# Autodesk Inventor assembly: Master
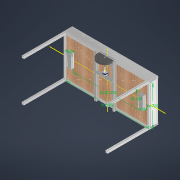
[picture p0: Inventor's stored thumbnail of the model, 180x180]
Saved by Autodesk Inventor 2021.4 (Build 254397000, 397)
## iProperties
Created: 2021-11-23
Part Number: Master
Document SubType Name: Assembly
Designer: jo_ki
Author: jo_ki
## Documents named in this file (34)
- D:\Repos\SmartSoccerTableCAD\Assemblies\Master.iam
- D:\Repos\SmartSoccerTableCAD\Parts\Beams\leg.ipt
- D:\Repos\SmartSoccerTableCAD\Parts\Beams\tallBeamLong.ipt
- D:\Repos\SmartSoccerTableCAD\Parts\Beams\tallBeamShort.ipt
- D:\Repos\SmartSoccerTableCAD\Parts\Beams\tallBeamLongInlet.ipt
- D:\Repos\SmartSoccerTableCAD\Parts\ballInlet\ballInletWheel.ipt
- D:\Repos\SmartSoccerTableCAD\Parts\Dimensions\Mastersketch.ipt
- D:\Repos\SmartSoccerTableCAD\Parts\Floors\GroundPlate.ipt
- D:\Repos\SmartSoccerTableCAD\Parts\Floors\glassPlate.ipt
- D:\Repos\SmartSoccerTableCAD\Parts\goalStructure\goalPanelFront.ipt
- D:\Repos\SmartSoccerTableCAD\Parts\goalStructure\goalPanelTop.ipt
- D:\Repos\SmartSoccerTableCAD\Parts\Beams\centerSupportBeam.ipt
- D:\Repos\SmartSoccerTableCAD\Import\stepper_am23hs0420-01\stepper_am23hs0420-01.iam
- D:\Repos\SmartSoccerTableCAD\Parts\Beams\centerAxleSupportBeam.ipt
- D:\Repos\SmartSoccerTableCAD\Parts\ballInlet\stepperMotorMount.ipt
- D:\Repos\SmartSoccerTableCAD\Parts\Beams\centerAxleSupportBeamHole.ipt
- D:\Repos\SmartSoccerTableCAD\Parts\ballInlet\axleMount\bearingShellInner.ipt
- D:\Repos\SmartSoccerTableCAD\Parts\ballInlet\axleMount\bearingShellOuter.ipt
- D:\Repos\SmartSoccerTableCAD\Parts\ballInlet\axleMount\centerAxleBearingSpacer.ipt
- D:\Repos\SmartSoccerTableCAD\Content Center Files\en-US\DIN 625 SKF(4)\DIN 625 SKF - SKF 61800-2Z.ipt
- D:\Repos\SmartSoccerTableCAD\Parts\ballInlet\ballInletWheelAxle.ipt
- D:\Repos\SmartSoccerTableCAD\Parts\ballInlet\stepperToAxleConnector_1.ipt
- D:\Repos\SmartSoccerTableCAD\Parts\ballInlet\stepperToAxleConnector_2.ipt
- D:\Repos\SmartSoccerTableCAD\Content Center Files\en-US\ISO 4762(2)\ISO 4762 - M3 x 6ISO.ipt
- D:\Repos\SmartSoccerTableCAD\Content Center Files\en-US\ISO 4762(2)\ISO 4762 - M5 x 16ISO.ipt
- D:\Repos\SmartSoccerTableCAD\Content Center Files\en-US\ISO 4035(2)\ISO 4035 - M10 - ISO.ipt
- D:\Repos\SmartSoccerTableCAD\Content Center Files\en-US\ISO 7089\ISO 7089 - 10 - 140 HV(1).ipt
- D:\Repos\SmartSoccerTableCAD\Import\Nutenstein_8_St_M6\Nutenstein_8_St_M6.ipt
- D:\Repos\SmartSoccerTableCAD\Content Center Files\en-US\ISO 4762(2)\ISO 4762 - M6 x 16ISO.ipt
- D:\Repos\SmartSoccerTableCAD\Parts\goalStructure\TorraumSeitenplatte.ipt
- D:\Repos\SmartSoccerTableCAD\Parts\goalStructure\TorraumSchrägeOben.ipt
- D:\Repos\SmartSoccerTableCAD\Parts\goalStructure\TorraumHinten.ipt
- D:\Repos\SmartSoccerTableCAD\Parts\goalStructure\TorraumFrontKlein.ipt
- D:\Repos\SmartSoccerTableCAD\Parts\goalStructure\goalPanelBottomSlope.ipt
## Components (53 placed, 32 different names)
1. glassPlate:1 — Mate:15, Mate:16, Flush:29, Mate:19, Mate:21
2. GroundPlate:1 — Mate:10, Mate:11, Mate:12, Mate:15, Flush:29, Mate:18, Mate:22, Mate:26, Mate:85, Mate:125
3. Nutenstein_8_St_M6:1 — Mate:80, Mate:81, Mate:82, Mate:83
4. ISO 4762 M6 x 16:1 — Mate:83, Mate:84
5. ISO 4762 M3 x 6:5 — Mate:62, Mate:63
6. ISO 4762 M3 x 6:6 — Mate:64, Mate:65
7. ISO 4762 M3 x 6:7 — Mate:66, Mate:67
8. ISO 4762 M5 x 16:5 — Mate:68, Mate:69
9. ISO 4762 M5 x 16:6 — Mate:70, Mate:71
10. ISO 4762 M5 x 16:7 — Mate:72, Mate:73
11. ISO 4762 M5 x 16:8 — Mate:74, Mate:75
12. ISO 7089 10:1 — Mate:76, Mate:77, Mate:79
13. ISO 4035 M10:1 — Mate:78, Mate:79, Angle:1
14. stepper_am23hs0420-01:1 [sub-assembly] — Flush:37, Mate:36, Mate:37, Mate:69, Mate:71, Mate:73, Mate:75
15. stepperMotorMount:1 — Mate:34, Mate:35, Flush:37, Mate:37, Mate:68, Mate:70, Mate:72, Mate:74, Mate:81, Mate:82, Mate:84
16. centerAxleSupportBeamHole:1 — Mate:38, Mate:39, Mate:40, Mate:41, Mate:50, Mate:51
17. bearingShellInner:1 — Mate:42, Mate:43, Mate:44, Mate:45, Mate:47
18. bearingShellOuter:1 — Mate:42, Mate:46, Mate:50, Mate:51
19. centerAxleBearingSpacer:1 — Mate:47, Mate:48, Mate:49
20. DIN 625 SKF- with two Z shields SKF 61800-2Z:3 — Mate:43, Mate:44, Mate:49
21. DIN 625 SKF- with two Z shields SKF 61800-2Z:4 — Mate:45, Mate:46, Mate:48
22. ballInletWheelAxle:1 — Mate:52, Mate:53, Mate:54, Mate:55, Mate:56, Mate:57, Mate:59, Mate:76, Mate:78, Angle:1
23. stepperToAxleConnector_1:1 — Flush:38, Mate:58, Mate:59, Mate:61, Mate:63, Mate:65, Mate:67
24. stepperToAxleConnector_2:1 — Mate:55, Mate:56, Mate:57, Flush:38, Mate:58, Mate:60, Mate:62, Mate:64, Mate:66
25. ISO 4762 M3 x 6:8 — Mate:60, Mate:61
26. centerSupportBeam:1 — Mate:29, Flush:32, Tangent:2, Mate:32, Flush:35, Mate:38
27. centerSupportBeam:2 — Mate:30, Flush:33, Tangent:1
28. centerAxleSupportBeam:1 — Mate:32, Flush:35, Mate:34, Mate:35, Mate:41, Mate:80
29. ballInletWheel:1 — Mate:9, Flush:17, Tangent:1, Tangent:2, Mate:36, Mate:39, Mate:40, Mate:52, Mate:53, Mate:54, Mate:77
30. leg:1 — Flush:1, Flush:23, Mate:14
31. leg:2 — Flush:14, Flush:15, Mate:8
32. leg:3 — Flush:3, Mate:13, Flush:21, Flush:22
33. leg:4 — Mate:6, Flush:12, Flush:13
34. tallBeamLong:1 — Flush:1, Flush:3, Mate:3, Mate:5, Mate:11, Flush:18, Flush:19, Flush:20, Mate:13, Flush:21, Mate:14, Mate:17, Mate:20, Mate:23, Mate:25
35. tallBeamShort:1 — Mate:5, Flush:15, Flush:16, Flush:20, Flush:22
36. tallBeamShort:2 — Mate:3, Flush:10, Mate:7, Flush:11, Flush:12, Mate:12, Flush:18, Flush:19, Flush:23
37. tallBeamLongInlet:1 — Mate:6, Flush:10, Mate:7, Flush:11, Flush:13, Flush:14, Flush:16, Mate:8, Mate:9, Flush:17, Mate:10, Mate:16, Mate:27, Mate:29, Flush:32, Mate:30, Flush:33
38. goalPanelFront:1 — Mate:17, Mate:18, Mate:19, Mate:26, Flush:31, Mate:28, Mate:86, Mate:88, Mate:90
39. TorraumSeitenplatte:1 — Mate:85, Mate:86, Mate:87, Mate:89, Flush:39, Flush:46, Mate:114, Mate:115
40. TorraumSeitenplatte:3 — Mate:116, Flush:47, Mate:117, Mate:119, Mate:127
41. TorraumSchrägeOben:1 — Mate:88, Mate:89, Mate:90, Mate:92
42. TorraumFrontKlein:1 — Flush:46, Mate:114, Mate:115, Mate:118
43. TorraumHinten:1 — Mate:91, Mate:92, Flush:39, Mate:116, Flush:47, Mate:117
44. goalPanelTop:1 — Mate:25, Mate:27, Flush:31, Mate:28, Mate:87, Mate:91
45. goalPanelBottomSlope:1 — Mate:118, Mate:119, Mate:127
46. goalPanelFront:2 — Mate:20, Mate:21, Mate:22, Mate:24, Flush:30, Flush:43, Mate:106, Mate:113
47. TorraumSeitenplatte:2 — Mate:110, Flush:45, Mate:111, Mate:126
48. TorraumSeitenplatte:4 — Mate:122, Flush:48, Flush:49, Mate:123, Mate:125, Flush:50, Mate:128
49. TorraumSchrägeOben:2 — Mate:112, Mate:113, Mate:126
50. TorraumFrontKlein:2 — Flush:43, Mate:106, Mate:122, Flush:48, Flush:49
51. TorraumHinten:2 — Mate:105, Mate:110, Flush:45, Mate:112, Mate:124, Flush:50
52. goalPanelTop:2 — Mate:23, Mate:24, Flush:30, Mate:105, Mate:111
53. goalPanelBottomSlope:2 — Mate:123, Mate:124, Mate:128
## Relationships (141: Mate 106, Flush 32, Tangent 2, Angle 1)
- Flush:1: leg:1 ↔ tallBeamLong:1
- Flush:3: leg:3 ↔ tallBeamLong:1
- Mate:3: tallBeamLong:1 ↔ tallBeamShort:2
- Mate:5: tallBeamLong:1 ↔ tallBeamShort:1
- Mate:6: leg:4 ↔ tallBeamLongInlet:1
- Flush:10: tallBeamShort:2 ↔ tallBeamLongInlet:1
- Mate:7: tallBeamShort:2 ↔ tallBeamLongInlet:1
- Flush:11: tallBeamShort:2 ↔ tallBeamLongInlet:1
- Flush:12: leg:4 ↔ tallBeamShort:2
- Flush:13: leg:4 ↔ tallBeamLongInlet:1
- Flush:14: leg:2 ↔ tallBeamLongInlet:1
- Flush:15: leg:2 ↔ tallBeamShort:1
- Flush:16: tallBeamShort:1 ↔ tallBeamLongInlet:1
- Mate:8: leg:2 ↔ tallBeamLongInlet:1
- Mate:9: ballInletWheel:1 ↔ tallBeamLongInlet:1
- Flush:17 (4.5 mm): ballInletWheel:1 ↔ tallBeamLongInlet:1
- Mate:10: GroundPlate:1 ↔ tallBeamLongInlet:1
- Mate:11 (-11 mm): GroundPlate:1 ↔ tallBeamLong:1
- Mate:12 (-11 mm): GroundPlate:1 ↔ tallBeamShort:2
- Flush:18: tallBeamLong:1 ↔ tallBeamShort:2
- Flush:19: tallBeamLong:1 ↔ tallBeamShort:2
- Flush:20: tallBeamLong:1 ↔ tallBeamShort:1
- Mate:13: leg:3 ↔ tallBeamLong:1
- Flush:21: leg:3 ↔ tallBeamLong:1
- Flush:22: leg:3 ↔ tallBeamShort:1
- Flush:23: leg:1 ↔ tallBeamShort:2
- Mate:14: leg:1 ↔ tallBeamLong:1
- Mate:15: glassPlate:1 ↔ GroundPlate:1
- Mate:16: glassPlate:1 ↔ tallBeamLongInlet:1
- Flush:29: glassPlate:1 ↔ GroundPlate:1
- Mate:17: tallBeamLong:1 ↔ goalPanelFront:1
- Mate:18: GroundPlate:1 ↔ goalPanelFront:1
- Mate:19: glassPlate:1 ↔ goalPanelFront:1
- Mate:20: tallBeamLong:1 ↔ goalPanelFront:2
- Mate:21: glassPlate:1 ↔ goalPanelFront:2
- Mate:22: GroundPlate:1 ↔ goalPanelFront:2
- Mate:23: tallBeamLong:1 ↔ goalPanelTop:2
- Mate:24: goalPanelFront:2 ↔ goalPanelTop:2
- Flush:30: goalPanelFront:2 ↔ goalPanelTop:2
- Mate:25: tallBeamLong:1 ↔ goalPanelTop:1
- Mate:26: GroundPlate:1 ↔ goalPanelFront:1
- Mate:27: tallBeamLongInlet:1 ↔ goalPanelTop:1
- Flush:31: goalPanelFront:1 ↔ goalPanelTop:1
- Mate:28: goalPanelFront:1 ↔ goalPanelTop:1
- Mate:29: centerSupportBeam:1 ↔ tallBeamLongInlet:1
- Flush:32: centerSupportBeam:1 ↔ tallBeamLongInlet:1
- Mate:30: centerSupportBeam:2 ↔ tallBeamLongInlet:1
- Flush:33: centerSupportBeam:2 ↔ tallBeamLongInlet:1
- Tangent:1 (10 mm): centerSupportBeam:2 ↔ ballInletWheel:1
- Tangent:2 (10 mm): centerSupportBeam:1 ↔ ballInletWheel:1
- Mate:32: centerSupportBeam:1 ↔ centerAxleSupportBeam:1
- Flush:35: centerSupportBeam:1 ↔ centerAxleSupportBeam:1
- Mate:34: stepperMotorMount:1 ↔ centerAxleSupportBeam:1
- Mate:35: stepperMotorMount:1 ↔ centerAxleSupportBeam:1
- Flush:37: stepper_am23hs0420-01:1 ↔ stepperMotorMount:1
- Mate:36: stepper_am23hs0420-01:1 ↔ ballInletWheel:1
- Mate:37: stepper_am23hs0420-01:1 ↔ stepperMotorMount:1
- Mate:38: centerAxleSupportBeamHole:1 ↔ centerSupportBeam:1
- Mate:39: centerAxleSupportBeamHole:1 ↔ ballInletWheel:1
- Mate:40 (10 mm): centerAxleSupportBeamHole:1 ↔ ballInletWheel:1
- Mate:41 (200 mm): centerAxleSupportBeamHole:1 ↔ centerAxleSupportBeam:1
- Mate:42: bearingShellInner:1 ↔ bearingShellOuter:1
- Mate:43: bearingShellInner:1 ↔ DIN 625 SKF- with two Z shields SKF 61800-2Z:3
- Mate:44: bearingShellInner:1 ↔ DIN 625 SKF- with two Z shields SKF 61800-2Z:3
- Mate:45: bearingShellInner:1 ↔ DIN 625 SKF- with two Z shields SKF 61800-2Z:4
- Mate:46: bearingShellOuter:1 ↔ DIN 625 SKF- with two Z shields SKF 61800-2Z:4
- Mate:47: bearingShellInner:1 ↔ centerAxleBearingSpacer:1
- Mate:48: centerAxleBearingSpacer:1 ↔ DIN 625 SKF- with two Z shields SKF 61800-2Z:4
- Mate:49: centerAxleBearingSpacer:1 ↔ DIN 625 SKF- with two Z shields SKF 61800-2Z:3
- Mate:50: centerAxleSupportBeamHole:1 ↔ bearingShellOuter:1
- Mate:51: centerAxleSupportBeamHole:1 ↔ bearingShellOuter:1
- Mate:52: ballInletWheelAxle:1 ↔ ballInletWheel:1
- Mate:53: ballInletWheelAxle:1 ↔ ballInletWheel:1
- Mate:54: ballInletWheelAxle:1 ↔ ballInletWheel:1
- Mate:55: ballInletWheelAxle:1 ↔ stepperToAxleConnector_2:1
- Mate:56: ballInletWheelAxle:1 ↔ stepperToAxleConnector_2:1
- Mate:57 (2.5 mm): ballInletWheelAxle:1 ↔ stepperToAxleConnector_2:1
- Flush:38: stepperToAxleConnector_1:1 ↔ stepperToAxleConnector_2:1
- Mate:58: stepperToAxleConnector_1:1 ↔ stepperToAxleConnector_2:1
- Mate:59: ballInletWheelAxle:1 ↔ stepperToAxleConnector_1:1
- Mate:60: stepperToAxleConnector_2:1 ↔ ISO 4762 M3 x 6:8
- Mate:61: stepperToAxleConnector_1:1 ↔ ISO 4762 M3 x 6:8
- Mate:62: ISO 4762 M3 x 6:5 ↔ stepperToAxleConnector_2:1
- Mate:63: ISO 4762 M3 x 6:5 ↔ stepperToAxleConnector_1:1
- Mate:64: ISO 4762 M3 x 6:6 ↔ stepperToAxleConnector_2:1
- Mate:65: ISO 4762 M3 x 6:6 ↔ stepperToAxleConnector_1:1
- Mate:66: ISO 4762 M3 x 6:7 ↔ stepperToAxleConnector_2:1
- Mate:67: ISO 4762 M3 x 6:7 ↔ stepperToAxleConnector_1:1
- Mate:68: ISO 4762 M5 x 16:5 ↔ stepperMotorMount:1
- Mate:69: ISO 4762 M5 x 16:5 ↔ stepper_am23hs0420-01:1
- Mate:70: ISO 4762 M5 x 16:6 ↔ stepperMotorMount:1
- Mate:71: ISO 4762 M5 x 16:6 ↔ stepper_am23hs0420-01:1
- Mate:72: ISO 4762 M5 x 16:7 ↔ stepperMotorMount:1
- Mate:73: ISO 4762 M5 x 16:7 ↔ stepper_am23hs0420-01:1
- Mate:74: ISO 4762 M5 x 16:8 ↔ stepperMotorMount:1
- Mate:75: ISO 4762 M5 x 16:8 ↔ stepper_am23hs0420-01:1
- Mate:76: ISO 7089 10:1 ↔ ballInletWheelAxle:1
- Mate:77: ISO 7089 10:1 ↔ ballInletWheel:1
- Mate:78: ISO 4035 M10:1 ↔ ballInletWheelAxle:1
- Mate:79: ISO 7089 10:1 ↔ ISO 4035 M10:1
- Angle:1 (0 deg): ISO 4035 M10:1 ↔ ballInletWheelAxle:1
- Mate:80: Nutenstein_8_St_M6:1 ↔ centerAxleSupportBeam:1
- Mate:81: Nutenstein_8_St_M6:1 ↔ stepperMotorMount:1
- Mate:82 (1 mm): Nutenstein_8_St_M6:1 ↔ stepperMotorMount:1
- Mate:83: Nutenstein_8_St_M6:1 ↔ ISO 4762 M6 x 16:1
- Mate:84: ISO 4762 M6 x 16:1 ↔ stepperMotorMount:1
- Mate:85: GroundPlate:1 ↔ TorraumSeitenplatte:1
- Mate:86: goalPanelFront:1 ↔ TorraumSeitenplatte:1
- Mate:87: TorraumSeitenplatte:1 ↔ goalPanelTop:1
- Mate:88: goalPanelFront:1 ↔ TorraumSchrägeOben:1
- Mate:89: TorraumSeitenplatte:1 ↔ TorraumSchrägeOben:1
- Mate:90: goalPanelFront:1 ↔ TorraumSchrägeOben:1
- Mate:91: TorraumHinten:1 ↔ goalPanelTop:1
- Mate:92: TorraumSchrägeOben:1 ↔ TorraumHinten:1
- Flush:39: TorraumSeitenplatte:1 ↔ TorraumHinten:1
- Mate:105: TorraumHinten:2 ↔ goalPanelTop:2
- Flush:43: goalPanelFront:2 ↔ TorraumFrontKlein:2
- Mate:106: goalPanelFront:2 ↔ TorraumFrontKlein:2
- Mate:110: TorraumSeitenplatte:2 ↔ TorraumHinten:2
- Flush:45: TorraumSeitenplatte:2 ↔ TorraumHinten:2
- Mate:111: TorraumSeitenplatte:2 ↔ goalPanelTop:2
- Mate:112: TorraumSchrägeOben:2 ↔ TorraumHinten:2
- Mate:113: goalPanelFront:2 ↔ TorraumSchrägeOben:2
- Flush:46: TorraumSeitenplatte:1 ↔ TorraumFrontKlein:1
- Mate:114: TorraumSeitenplatte:1 ↔ TorraumFrontKlein:1
- Mate:115: TorraumSeitenplatte:1 ↔ TorraumFrontKlein:1
- Mate:116: TorraumSeitenplatte:3 ↔ TorraumHinten:1
- Flush:47: TorraumSeitenplatte:3 ↔ TorraumHinten:1
- Mate:117: TorraumSeitenplatte:3 ↔ TorraumHinten:1
- Mate:118: TorraumFrontKlein:1 ↔ goalPanelBottomSlope:1
- Mate:119: TorraumSeitenplatte:3 ↔ goalPanelBottomSlope:1
- Mate:122: TorraumSeitenplatte:4 ↔ TorraumFrontKlein:2
- Flush:48: TorraumSeitenplatte:4 ↔ TorraumFrontKlein:2
- Flush:49: TorraumSeitenplatte:4 ↔ TorraumFrontKlein:2
- Mate:123: TorraumSeitenplatte:4 ↔ goalPanelBottomSlope:2
- Mate:124: TorraumHinten:2 ↔ goalPanelBottomSlope:2
- Mate:125: GroundPlate:1 ↔ TorraumSeitenplatte:4
- Flush:50: TorraumSeitenplatte:4 ↔ TorraumHinten:2
- Mate:126: TorraumSeitenplatte:2 ↔ TorraumSchrägeOben:2
- Mate:127: TorraumSeitenplatte:3 ↔ goalPanelBottomSlope:1
- Mate:128: TorraumSeitenplatte:4 ↔ goalPanelBottomSlope:2
## Named parameters: profile_width = 40 mm, feet_widthCenter = 720 mm, feet_lengthCenter = 1500 mm, feet_length = 746 mm, profile_height = 160 mm, groundPlate_width = 702 mm, groundPlate_length = 1482 mm, handle_distance = 150 mm, handle_amount = 8, handle_offsetTop = 45 mm, handleAxle_diameter = 16 mm, handleHole_diameter = 36 mm, profileTall_innerHeightOffset = 33 mm, profileTallWall_thickness = 3 mm, groundPlate_thickness = 8 mm, ball_size = 33 mm, ball_rollTolerance = 1 mm, glass_thickness = 6 mm, glass_length = 1200 mm, ballInletHole_groundPlateOffsetBottom = 24 mm, ballInletWheel_margin = 10 mm, ballInletWheel_thickness = 31 mm, ballInletWheelBucket_amount = 6, ballInletWheelSlope_angle = 10 deg, goal_width = 224 mm, goal_height = 96 mm, goal_depth = 84 mm, goalCollector_depth = 68 mm, ballRollbackRail_angle = 7 deg, handleAxle_length = 1100 mm, ballInletWheelDriveShaftAxle_diameter = 10 mm, ballInletWheel_diameter = 265.32266 mm, ballInletWheel_offsetTop = 185.19519 mm, ballInletWheel_tolerance = 1 mm, ballInletHole_bottomOffset = 73 mm, playAreaWall_height = 130 mm, goalPanel_thickness = 4 mm, goalArea_width = 130 mm, goalCollector_angle = 45 deg, goalCollectorRollback_angle = 45 deg, goalPlayArea_distance = 228 mm, goalPanelFrontInner_innerWidth = 220 mm, goalPanelBackInner_innerWidth = 672 mm, goalPanelSideOuter_width = 141 mm, goalCollectorPanelSide_angel = 45 deg, pipeConnector_wallThickness = 3 mm, pipe_wallThickness = 2 mm, axleSupport_offset = 25.19519 mm, axleSupport_distance = 200 mm
